# Autodesk Inventor assembly: 新款四方轴套_MIR
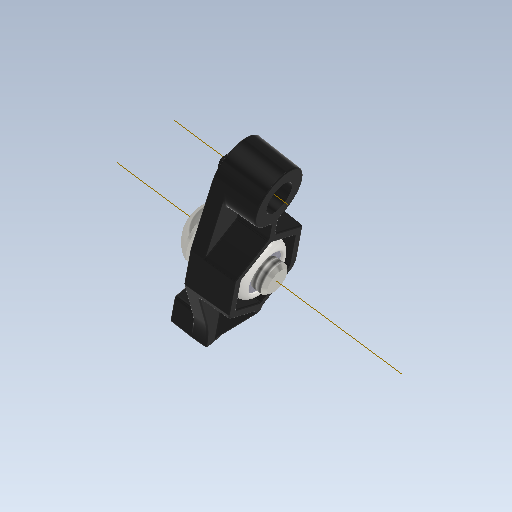
[picture p0: Inventor's stored thumbnail of the model, 512x512]
Saved by Autodesk Inventor 2020 (Build 240168000, 168)
## iProperties
Created: 2019-05-29
Part Number: 新款四方轴套_MIR
Document SubType Name: Assembly
Designer: 31144
Author: aresp
## Documents named in this file (4)
- C:\Users\31144\Documents\Vault\ncrCadLib\轴相关\细轴配套\新款四方轴套_MIR.iam
- C:\Users\31144\Documents\Vault\ncrCadLib\轴相关\细轴配套\零件\细轴新款四方轴承_MIR.ipt
- C:\Users\31144\Documents\Vault\ncrCadLib\螺丝螺帽\Screw 8-32 x 0.375'' 二号_MIR.ipt
- C:\Users\31144\Documents\Vault\ncrCadLib\螺丝螺帽\防滑螺帽_MIR.ipt
## Components (3 placed, 3 different names)
1. 细轴新款四方轴承_MIR:1 — 配合:5, 配合:4
2. Screw 8-32 x 0.375'' 二号_MIR:1 — 配合:5, 配合:4, 配合:2, 配合:1
3. 防滑螺帽_MIR:1 — 配合:2, 配合:1
## Relationships (4: Mate 4)
- 配合:5 [Mate] (1.5748 mm): 细轴新款四方轴承_MIR:1 ↔ Screw 8-32 x 0.375'' 二号_MIR:1
- 配合:4 [Mate]: 细轴新款四方轴承_MIR:1 ↔ Screw 8-32 x 0.375'' 二号_MIR:1
- 配合:2 [Mate] (3.1242 mm): Screw 8-32 x 0.375'' 二号_MIR:1 ↔ 防滑螺帽_MIR:1
- 配合:1 [Mate]: Screw 8-32 x 0.375'' 二号_MIR:1 ↔ 防滑螺帽_MIR:1
